# Autodesk Inventor assembly: assembled
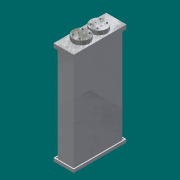
[picture p0: Inventor's stored thumbnail of the model, 180x180]
Saved by Autodesk Inventor 2016 (Build 200138000, 138)
## iProperties
Created: 2016-07-15
Part Number: assembled
Document SubType Name: Assembly
Designer: Jonathan
Author: Jonathan
## Documents named in this file (6)
- C:\Users\sawaiz\oneDrive\projects\neutronCell\neutronCell.iam
- C:\Users\sawaiz\oneDrive\projects\neutronCell\blankCap.ipt
- C:\Users\sawaiz\oneDrive\projects\neutronCell\tube.ipt
- C:\Users\sawaiz\oneDrive\projects\neutronCell\sensorCap.ipt
- C:\Users\sawaiz\oneDrive\projects\neutronCell\sensorHolder.iam
- C:\Users\sawaiz\oneDrive\projects\neutronCell\parameters.xlsx
## Components (5 placed, 4 different names)
1. blankCap:1 — Mate:2, Mate:3, Mate:4, Flush:1, Flush:2
2. tube:1 — Mate:1, Mate:2, Mate:3, Mate:4
3. sensorCap:1 — Mate:1, Flush:1, Flush:2, Mate:5, Mate:6, Mate:7
4. sensorHolder:1 [sub-assembly] — Mate:5, Mate:6, Mate:7
5. sensorHolder:2 [sub-assembly]
## Component patterns: (2 elements, first: sensorHolder:1)
## Relationships (9: Mate 7, Flush 2)
- Mate:1: tube:1 ↔ sensorCap:1
- Mate:2: blankCap:1 ↔ tube:1
- Mate:3 (0.127 mm): blankCap:1 ↔ tube:1
- Mate:4 (0.127 mm): blankCap:1 ↔ tube:1
- Flush:1: blankCap:1 ↔ sensorCap:1
- Flush:2: blankCap:1 ↔ sensorCap:1
- Mate:5: sensorCap:1 ↔ sensorHolder:1
- Mate:6: sensorCap:1 ↔ sensorHolder:1
- Mate:7: sensorCap:1 ↔ sensorHolder:1
## Named parameters: tubeHeight = 50.8 mm, tubeWidth = 152.4 mm, tubeLength = 304.8 mm, tubeWallThickness = 3.175 mm, plateOverhang = 6.35 mm, moatWidth = 3.175 mm, moatDepth = 3.175 mm, tubePlateClearance = 0.127 mm, blankCapThickness = 9.525 mm, sensorCapThickness = 12.7 mm, glassTubeDiameter = 12.7 mm, glassTubeClearance = 0.19844 mm, sensorHoles = 2, longHoleSpacing = 30.48 mm, shortHoleSpacing = 21.59 mm, sensorHolderDiameter = 50.8 mm, sensorHolderThickness = 12.7 mm, fiberDiameter = 1 mm, fiberClearance = 0 mm, oRingID = 22.2504 mm, oRingGrooveWidth = 2.54 mm, oRingGrooveDepth = 1.2446 mm, glassTubeLength = 279.4 mm, glassTubeID = 7.874 mm, sensorBoardHoleSpacing = 19 mm
